# Autodesk Inventor assembly: GlyphPlate
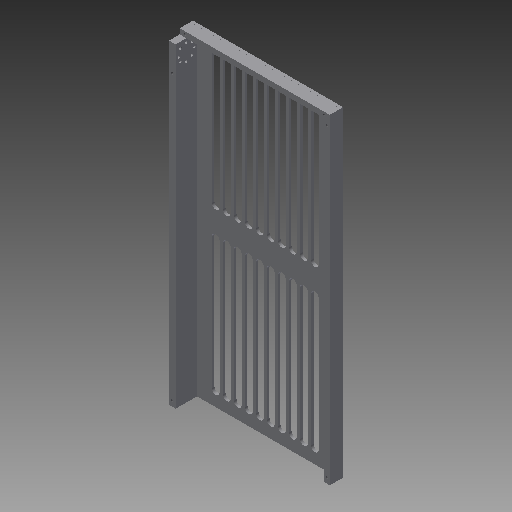
[picture p0: Inventor's stored thumbnail of the model, 512x512]
Saved by Autodesk Inventor 2017 (Build 210142000, 142)
## iProperties
Created: 2018-01-27
Part Number: GlyphPlate
Document SubType Name: Assembly
Designer: User
Author: User
## Documents named in this file (5)
- C:\Robotics\CAD\2017-18_CAD\GlyphPlate.iam
- C:\Robotics\CAD\2017-18_CAD\GlyphPlateBackSide.ipt
- C:\Robotics\CAD\2017-18_CAD\GlyphPlateLeftSide.ipt
- C:\Robotics\CAD\2017-18_CAD\GlyphPlateRightSide.ipt
- C:\Robotics\CAD\2017-18_CAD\GlyphPlateUnderside.ipt
## Components (4 placed, 4 different names)
1. GlyphPlateBackSide:1 — Mate:1, Flush:1, Mate:2, Flush:3, Flush:5, Mate:4
2. GlyphPlateLeftSide:1 — Mate:2, Flush:3, Mate:3
3. GlyphPlateRightSide:1 — Mate:1, Flush:1, Flush:6, Mate:5
4. GlyphPlateUnderside:1 — Flush:5, Flush:6, Mate:3, Mate:4, Mate:5
## Relationships (9: Mate 5, Flush 4)
- Mate:1: GlyphPlateBackSide:1 ↔ GlyphPlateRightSide:1
- Flush:1: GlyphPlateBackSide:1 ↔ GlyphPlateRightSide:1
- Mate:2: GlyphPlateBackSide:1 ↔ GlyphPlateLeftSide:1
- Flush:3: GlyphPlateBackSide:1 ↔ GlyphPlateLeftSide:1
- Flush:5: GlyphPlateBackSide:1 ↔ GlyphPlateUnderside:1
- Flush:6: GlyphPlateRightSide:1 ↔ GlyphPlateUnderside:1
- Mate:3: GlyphPlateLeftSide:1 ↔ GlyphPlateUnderside:1
- Mate:4: GlyphPlateBackSide:1 ↔ GlyphPlateUnderside:1
- Mate:5: GlyphPlateRightSide:1 ↔ GlyphPlateUnderside:1
